# Autodesk Inventor assembly: Electric Flipper V1
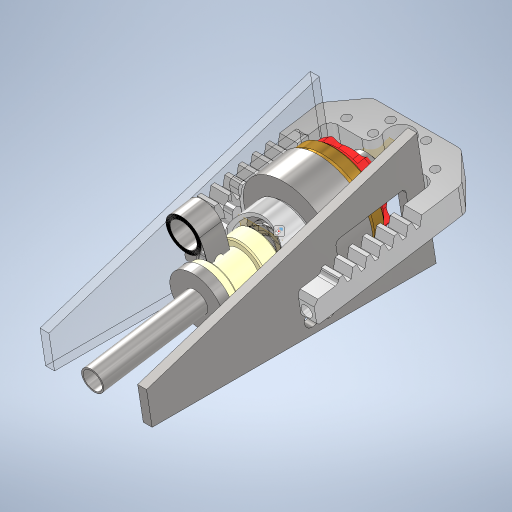
[picture p0: Inventor's stored thumbnail of the model, 512x512]
Saved by Autodesk Inventor 2023.2 (Build 272271000, 271)
## iProperties
Created: 2024-03-17
Part Number: Electric Flipper V1
Document SubType Name: Assembly
Designer: Nathan Cai
Mass: 282.609 g
Surface Area: 532.175 cm^2
Volume: 45.1635 cm^3
Density: 6.25747 g/cm^3
Author: Nathan Cai
## Documents named in this file (16)
- E:\Documents\Inventor\Bleep V2\Electric Flipper V1.iam
- E:\Documents\Inventor\Bleep V2\AKK RS2205 2300KV\AKK RS2205 2300KV.iam
- E:\Documents\Inventor\Bleep V2\Flywheel.ipt
- E:\Documents\Inventor\Bleep V2\Clutch.ipt
- E:\Documents\Inventor\Bleep V2\Shaft.ipt
- E:\Documents\Inventor\Bleep V2\BB 13x19x4.ipt
- E:\Documents\Inventor\Bleep V2\Cup.ipt
- E:\Documents\Inventor\Bleep V2\1561T741_Stacked Wave Disc Spring\1561T741_Stacked Wave Disc Spring.ipt
- E:\Documents\Inventor\Bleep V2\Spring Anchor.ipt
- E:\Documents\Inventor\Bleep V2\9293K44_Constant-Force Spring\9293K44_Constant-Force Spring.ipt
- E:\Documents\Inventor\Bleep V2\BB 5-16x 1-2x 5-32in - Flangeless.ipt
- E:\Documents\Inventor\Bleep V2\Thrust Bearing.ipt
- E:\Documents\Inventor\Bleep V2\Upright.ipt
- E:\Documents\Inventor\Bleep V2\Rack.ipt
- E:\Documents\Inventor\Bleep V2\Lever.ipt
- E:\Documents\Inventor\Bleep V2\BB 3x7x4.ipt
## Components (17 placed, 15 different names)
1. AKK RS2205 2300KV:1 [sub-assembly] — Mate:1, Flush:1, Mate:3, Mate:22, Mate:23, Mate:26
2. Flywheel:1 — Mate:1, Flush:1, Mate:2, Mate:5, Mate:20
3. Clutch:1 — Mate:2, Mate:4, Mate:8, Mate:9
4. Shaft:1 — Mate:3, Mate:4, Mate:5, Mate:10, Flush:3, Flush:4, Mate:15, Mate:16, Mate:17, Mate:19, Mate:21, Mate:24, Mate:26, Flush:6, Mate:28, Mate:33
5. BB 13x19x4:1 — Mate:6, Mate:7, Mate:8, Mate:9
6. Cup:1 — Mate:6, Mate:7, Tangent:1, Mate:33
7. 1561T741_Stacked Wave Disc Spring:1 — Mate:10, Flush:4
8. Spring Anchor:1 — Mate:15, Mate:16, Mate:18, Mate:27
9. 9293K44_Constant-Force Spring:1 — Mate:27
10. BB 5-16x 1-2x 5-32in - Flangeless:1 — Mate:19, Mate:20
11. Thrust Bearing:1 — Mate:17, Mate:18
12. BB 5-16x 1-2x 5-32in - Flangeless:2 — Mate:21, Mate:22
13. Upright:1 — Flush:5, Mate:23, Mate:24, Mate:25, Mate:29, Mate:30, Symmetry:1, Flush:7, Flush:8
14. Rack:1 — Flush:6, Mate:28
15. Lever:1 — Mate:29, Mate:30, Mate:31, Mate:32, Tangent:1
16. BB 3x7x4:1 — Mate:31, Mate:32
17. Upright:2 — Symmetry:1, Flush:7, Flush:8
## Relationships (38: Mate 29, Flush 7, Tangent 1, Symmetry 1)
- Mate:1: AKK RS2205 2300KV:1 ↔ Flywheel:1
- Flush:1: AKK RS2205 2300KV:1 ↔ Flywheel:1
- Mate:2: Flywheel:1 ↔ Clutch:1
- Mate:3: AKK RS2205 2300KV:1 ↔ Shaft:1
- Mate:4: Clutch:1 ↔ Shaft:1
- Mate:5: Flywheel:1 ↔ Shaft:1
- Mate:6: BB 13x19x4:1 ↔ Cup:1
- Mate:7: BB 13x19x4:1 ↔ Cup:1
- Mate:8: Clutch:1 ↔ BB 13x19x4:1
- Mate:9: Clutch:1 ↔ BB 13x19x4:1
- Mate:10: Shaft:1 ↔ 1561T741_Stacked Wave Disc Spring:1
- Flush:3: Shaft:1
- Flush:4: Shaft:1 ↔ 1561T741_Stacked Wave Disc Spring:1
- Mate:15: Shaft:1 ↔ Spring Anchor:1
- Mate:16: Shaft:1 ↔ Spring Anchor:1
- Mate:17: Shaft:1 ↔ Thrust Bearing:1
- Mate:18: Spring Anchor:1 ↔ Thrust Bearing:1
- Mate:19: Shaft:1 ↔ BB 5-16x 1-2x 5-32in - Flangeless:1
- Mate:20: Flywheel:1 ↔ BB 5-16x 1-2x 5-32in - Flangeless:1
- Mate:21: Shaft:1 ↔ BB 5-16x 1-2x 5-32in - Flangeless:2
- Mate:22 (0.7937 mm): AKK RS2205 2300KV:1 ↔ BB 5-16x 1-2x 5-32in - Flangeless:2
- Flush:5 (-15.875 mm): Upright:1
- Mate:23: AKK RS2205 2300KV:1 ↔ Upright:1
- Mate:24 (7.9375 mm): Shaft:1 ↔ Upright:1
- Mate:25: Upright:1
- Mate:26: AKK RS2205 2300KV:1 ↔ Shaft:1
- Mate:27: Spring Anchor:1 ↔ 9293K44_Constant-Force Spring:1
- Flush:6: Shaft:1 ↔ Rack:1
- Mate:28: Shaft:1 ↔ Rack:1
- Mate:29: Upright:1 ↔ Lever:1
- Mate:30: Upright:1 ↔ Lever:1
- Mate:31: Lever:1 ↔ BB 3x7x4:1
- Mate:32 (3.175 mm): Lever:1 ↔ BB 3x7x4:1
- Tangent:1: Cup:1 ↔ Lever:1
- Mate:33: Shaft:1 ↔ Cup:1
- Symmetry:1: Upright:1 ↔ Upright:2
- Flush:7: Upright:1 ↔ Upright:2
- Flush:8: Upright:1 ↔ Upright:2
